# Autodesk Inventor assembly: Chassis
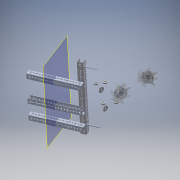
[picture p0: Inventor's stored thumbnail of the model, 180x180]
Saved by Autodesk Inventor 2018 (Build 220112000, 112)
## iProperties
Created: 2017-11-01
Part Number: Chassis
Document SubType Name: Assembly
Designer: Kitte
Author: Kitte
## Documents named in this file (9)
- C:\Users\Kitte\Documents\GitHub\7729-CAD\2017-18_CAD\Chassis.iam
- C:\Users\Kitte\Documents\Git\Robotics\lib\Tetrix\Structural_components\Channel 288mm.ipt
- C:\Users\Kitte\Documents\GitHub\7729-CAD\2017-18_CAD\Channel416mm_BearingHoles.ipt
- C:\Users\Kitte\Documents\GitHub\7729-CAD\lib\AndyMark\Misc\am-3377+6x12x4+Flanged+Bearing.ipt
- C:\Users\Kitte\Documents\GitHub\7729-CAD\lib\AndyMark\Misc\am-3226-100+6mm+D-Shaft+100mm.ipt
- C:\Users\Kitte\Documents\GitHub\7729-CAD\lib\Tetrix\Axels_hubs_and_collars\Motor Shaft (6mm) Hub.ipt
- C:\Users\Kitte\Documents\GitHub\7729-CAD\lib\Tetrix\Gears_and_sprockets\Gear 40 Tooth.ipt
- C:\Users\Kitte\Documents\GitHub\7729-CAD\lib\Tetrix\Gears_and_sprockets\am-2538 - 4 in mecanum left wheel.ipt
- C:\Users\Kitte\Documents\GitHub\7729-CAD\lib\Tetrix\Gears_and_sprockets\am-2538 - 4 in mecanum right wheel.ipt
## Components (22 placed, 8 different names)
1. Channel 288mm:1 — Mate:10, Mate:11
2. Channel 288mm:2 — Mate:5, Mate:6
3. Channel 288mm:3 — Mate:7, Mate:8, Mate:26
4. Channel416mm_BearingHoles:1 — Mate:5, Mate:6, Mate:7, Mate:8, Mate:10, Mate:11, Insert:3, Insert:4, Insert:7, Insert:8, Angle:5
5. am-3377+6x12x4+Flanged+Bearing:1 — Insert:8, Mate:13, Mate:16
6. am-3377+6x12x4+Flanged+Bearing:2 — Insert:7, Mate:12, Mate:22
7. am-3377+6x12x4+Flanged+Bearing:5 — Insert:4, Mate:18, Mate:20
8. am-3377+6x12x4+Flanged+Bearing:6 — Insert:3, Mate:21, Mate:24
9. am-3226-100+6mm+D-Shaft+100mm:1 — Mate:12, Mate:21, Mate:23, Angle:3, Mate:25, Angle:4
10. am-3226-100+6mm+D-Shaft+100mm:4 — Mate:13, Mate:17, Mate:19, Angle:1, Angle:2, Mate:20
11. Motor Shaft (6mm) Hub:1 — Mate:24, Mate:25, Angle:4
12. Motor Shaft (6mm) Hub:4 — Mate:18, Mate:19, Angle:2
13. Motor Shaft (6mm) Hub:5 — Mate:16, Mate:17, Angle:1
14. Motor Shaft (6mm) Hub:8 — Mate:22, Mate:23, Angle:3
15. Motor Shaft (6mm) Hub:9
16. Motor Shaft (6mm) Hub:10
17. Motor Shaft (6mm) Hub:11
18. Motor Shaft (6mm) Hub:12
19. Gear 40 Tooth:1
20. Gear 40 Tooth:2
21. am-2538 - 4 in mecanum left wheel:1
22. am-2538 - 4 in mecanum right wheel:1
## Relationships (28: Mate 19, Angle 5, Insert 4)
- Mate:5: Channel 288mm:2 ↔ Channel416mm_BearingHoles:1
- Mate:6: Channel 288mm:2 ↔ Channel416mm_BearingHoles:1
- Mate:7: Channel 288mm:3 ↔ Channel416mm_BearingHoles:1
- Mate:8: Channel 288mm:3 ↔ Channel416mm_BearingHoles:1
- Mate:10: Channel 288mm:1 ↔ Channel416mm_BearingHoles:1
- Mate:11: Channel 288mm:1 ↔ Channel416mm_BearingHoles:1
- Insert:3: Channel416mm_BearingHoles:1 ↔ am-3377+6x12x4+Flanged+Bearing:6
- Insert:4: Channel416mm_BearingHoles:1 ↔ am-3377+6x12x4+Flanged+Bearing:5
- Insert:7: Channel416mm_BearingHoles:1 ↔ am-3377+6x12x4+Flanged+Bearing:2
- Insert:8: Channel416mm_BearingHoles:1 ↔ am-3377+6x12x4+Flanged+Bearing:1
- Mate:12: am-3377+6x12x4+Flanged+Bearing:2 ↔ am-3226-100+6mm+D-Shaft+100mm:1
- Mate:13: am-3377+6x12x4+Flanged+Bearing:1 ↔ am-3226-100+6mm+D-Shaft+100mm:4
- Mate:16: am-3377+6x12x4+Flanged+Bearing:1 ↔ Motor Shaft (6mm) Hub:5
- Mate:17: am-3226-100+6mm+D-Shaft+100mm:4 ↔ Motor Shaft (6mm) Hub:5
- Mate:18: am-3377+6x12x4+Flanged+Bearing:5 ↔ Motor Shaft (6mm) Hub:4
- Mate:19: am-3226-100+6mm+D-Shaft+100mm:4 ↔ Motor Shaft (6mm) Hub:4
- Angle:1 (0 deg): am-3226-100+6mm+D-Shaft+100mm:4 ↔ Motor Shaft (6mm) Hub:5
- Angle:2 (0 deg): am-3226-100+6mm+D-Shaft+100mm:4 ↔ Motor Shaft (6mm) Hub:4
- Mate:20: am-3377+6x12x4+Flanged+Bearing:5 ↔ am-3226-100+6mm+D-Shaft+100mm:4
- Mate:21: am-3377+6x12x4+Flanged+Bearing:6 ↔ am-3226-100+6mm+D-Shaft+100mm:1
- Mate:22: am-3377+6x12x4+Flanged+Bearing:2 ↔ Motor Shaft (6mm) Hub:8
- Mate:23: am-3226-100+6mm+D-Shaft+100mm:1 ↔ Motor Shaft (6mm) Hub:8
- Angle:3 (0 deg): am-3226-100+6mm+D-Shaft+100mm:1 ↔ Motor Shaft (6mm) Hub:8
- Mate:24: am-3377+6x12x4+Flanged+Bearing:6 ↔ Motor Shaft (6mm) Hub:1
- Mate:25: am-3226-100+6mm+D-Shaft+100mm:1 ↔ Motor Shaft (6mm) Hub:1
- Angle:4 (0 deg): am-3226-100+6mm+D-Shaft+100mm:1 ↔ Motor Shaft (6mm) Hub:1
- Mate:26: Channel 288mm:3
- Angle:5 (0 deg): Channel416mm_BearingHoles:1
